# Autodesk Inventor assembly: robot base
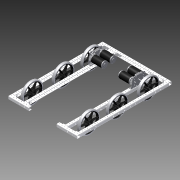
[picture p0: Inventor's stored thumbnail of the model, 180x180]
Saved by Autodesk Inventor 2011 SP1 (Build 150282100, 282)
## iProperties
Created: 2012-01-19
Part Number: robot base
Document SubType Name: Assembly
Designer: Christopher
Author: Christopher
## Documents named in this file (7)
- C:\Users\Christopher\Documents\Christopher\FIRST\Inventor files\2012\robot base.iam
- C:\Users\Christopher\Documents\Christopher\FIRST\Inventor files\2011\Kit of Parts\Chassis\Chassis_CornerConnect_AndyMark_am-0212.ipt
- C:\Users\Christopher\Documents\Christopher\FIRST\Inventor files\2011\Kit of Parts\Chassis\Chassis_CIMGearbox_AndyMark_am-0734.ipt
- C:\Users\Christopher\Documents\Christopher\FIRST\Inventor files\2011\Kit of Parts\Chassis\Chassis_Channel_AndyMark_am-0202.ipt
- C:\Users\Christopher\Documents\Christopher\FIRST\Inventor files\2011\Kit of Parts\Chassis\Chassis_Wheel_AndyMark_am-0420.iam
- C:\Users\Christopher\Documents\Christopher\FIRST\Inventor files\2011\Kit of Parts\Chassis\chassis 27 inch.ipt
- C:\Users\Christopher\Documents\Christopher\FIRST\Inventor files\2011\Kit of Parts\Chassis\chassis 9 inch.ipt
## Components (23 placed, 6 different names)
1. Chassis_CornerConnect_AndyMark_am-0212:1 — Insert:3, Insert:4, Insert:30
2. Chassis_CornerConnect_AndyMark_am-0212:4 — Insert:22, Insert:23, Insert:26, Insert:27
3. Chassis_CornerConnect_AndyMark_am-0212:5 — Insert:13, Insert:14, Insert:31
4. Chassis_CornerConnect_AndyMark_am-0212:6 — Insert:7, Insert:8
5. Chassis_CornerConnect_AndyMark_am-0212:7 — Insert:1, Insert:2, Insert:5, Insert:6
6. Chassis_CornerConnect_AndyMark_am-0212:8 — Insert:9, Insert:10, Insert:11, Insert:12
7. Chassis_CornerConnect_AndyMark_am-0212:9 — Insert:28, Insert:32
8. Chassis_CornerConnect_AndyMark_am-0212:10 — Insert:20, Insert:21, Insert:29
9. Chassis_CIMGearbox_AndyMark_am-0734:1 — Insert:35, Insert:36
10. Chassis_CIMGearbox_AndyMark_am-0734:2 — Insert:33, Insert:34
11. Chassis_Channel_AndyMark_am-0202:1 — Insert:11, Insert:12, Insert:13, Insert:14, Insert:37, Insert:38, Insert:39
12. Chassis_Channel_AndyMark_am-0202:3 — Insert:1, Insert:2, Insert:3, Insert:4, Insert:40, Insert:42, Insert:43
13. Chassis_Channel_AndyMark_am-0202:4 — Insert:26, Insert:27, Insert:28, Insert:33, Insert:34
14. Chassis_Channel_AndyMark_am-0202:5 — Insert:20, Insert:21, Insert:35, Insert:36
15. Chassis_Wheel_AndyMark_am-0420:1 [sub-assembly] — Insert:40
16. Chassis_Wheel_AndyMark_am-0420:2 [sub-assembly] — Insert:42
17. Chassis_Wheel_AndyMark_am-0420:3 [sub-assembly] — Insert:43
18. Chassis_Wheel_AndyMark_am-0420:4 [sub-assembly] — Insert:38
19. Chassis_Wheel_AndyMark_am-0420:5 [sub-assembly] — Insert:37
20. Chassis_Wheel_AndyMark_am-0420:6 [sub-assembly] — Insert:39
21. chassis 27 inch:1 — Insert:5, Insert:6, Insert:7, Insert:8, Insert:9, Insert:10, Insert:22, Insert:23
22. chassis 9 inch:1 — Insert:29, Insert:30
23. chassis 9 inch:2 — Insert:31, Insert:32
## Relationships (35: Insert 35)
- Insert:1: Chassis_CornerConnect_AndyMark_am-0212:7 ↔ Chassis_Channel_AndyMark_am-0202:3
- Insert:2: Chassis_CornerConnect_AndyMark_am-0212:7 ↔ Chassis_Channel_AndyMark_am-0202:3
- Insert:3: Chassis_CornerConnect_AndyMark_am-0212:1 ↔ Chassis_Channel_AndyMark_am-0202:3
- Insert:4: Chassis_CornerConnect_AndyMark_am-0212:1 ↔ Chassis_Channel_AndyMark_am-0202:3
- Insert:5: Chassis_CornerConnect_AndyMark_am-0212:7 ↔ chassis 27 inch:1
- Insert:6: Chassis_CornerConnect_AndyMark_am-0212:7 ↔ chassis 27 inch:1
- Insert:7: Chassis_CornerConnect_AndyMark_am-0212:6 ↔ chassis 27 inch:1
- Insert:8: Chassis_CornerConnect_AndyMark_am-0212:6 ↔ chassis 27 inch:1
- Insert:9: Chassis_CornerConnect_AndyMark_am-0212:8 ↔ chassis 27 inch:1
- Insert:10: Chassis_CornerConnect_AndyMark_am-0212:8 ↔ chassis 27 inch:1
- Insert:11: Chassis_CornerConnect_AndyMark_am-0212:8 ↔ Chassis_Channel_AndyMark_am-0202:1
- Insert:12: Chassis_CornerConnect_AndyMark_am-0212:8 ↔ Chassis_Channel_AndyMark_am-0202:1
- Insert:13: Chassis_CornerConnect_AndyMark_am-0212:5 ↔ Chassis_Channel_AndyMark_am-0202:1
- Insert:14: Chassis_CornerConnect_AndyMark_am-0212:5 ↔ Chassis_Channel_AndyMark_am-0202:1
- Insert:20: Chassis_CornerConnect_AndyMark_am-0212:10 ↔ Chassis_Channel_AndyMark_am-0202:5
- Insert:21: Chassis_CornerConnect_AndyMark_am-0212:10 ↔ Chassis_Channel_AndyMark_am-0202:5
- Insert:22: Chassis_CornerConnect_AndyMark_am-0212:4 ↔ chassis 27 inch:1
- Insert:23: Chassis_CornerConnect_AndyMark_am-0212:4 ↔ chassis 27 inch:1
- Insert:26: Chassis_CornerConnect_AndyMark_am-0212:4 ↔ Chassis_Channel_AndyMark_am-0202:4
- Insert:27: Chassis_CornerConnect_AndyMark_am-0212:4 ↔ Chassis_Channel_AndyMark_am-0202:4
- Insert:28: Chassis_CornerConnect_AndyMark_am-0212:9 ↔ Chassis_Channel_AndyMark_am-0202:4
- Insert:29: Chassis_CornerConnect_AndyMark_am-0212:10 ↔ chassis 9 inch:1
- Insert:30: Chassis_CornerConnect_AndyMark_am-0212:1 ↔ chassis 9 inch:1
- Insert:31: Chassis_CornerConnect_AndyMark_am-0212:5 ↔ chassis 9 inch:2
- Insert:32: Chassis_CornerConnect_AndyMark_am-0212:9 ↔ chassis 9 inch:2
- Insert:33: Chassis_CIMGearbox_AndyMark_am-0734:2 ↔ Chassis_Channel_AndyMark_am-0202:4
- Insert:34: Chassis_CIMGearbox_AndyMark_am-0734:2 ↔ Chassis_Channel_AndyMark_am-0202:4
- Insert:35: Chassis_CIMGearbox_AndyMark_am-0734:1 ↔ Chassis_Channel_AndyMark_am-0202:5
- Insert:36: Chassis_CIMGearbox_AndyMark_am-0734:1 ↔ Chassis_Channel_AndyMark_am-0202:5
- Insert:37 (57.15 mm): Chassis_Channel_AndyMark_am-0202:1 ↔ Chassis_Wheel_AndyMark_am-0420:5
- Insert:38 (57.15 mm): Chassis_Channel_AndyMark_am-0202:1 ↔ Chassis_Wheel_AndyMark_am-0420:4
- Insert:39 (57.15 mm): Chassis_Channel_AndyMark_am-0202:1 ↔ Chassis_Wheel_AndyMark_am-0420:6
- Insert:40 (57.15 mm): Chassis_Channel_AndyMark_am-0202:3 ↔ Chassis_Wheel_AndyMark_am-0420:1
- Insert:42 (57.15 mm): Chassis_Channel_AndyMark_am-0202:3 ↔ Chassis_Wheel_AndyMark_am-0420:2
- Insert:43 (57.15 mm): Chassis_Channel_AndyMark_am-0202:3 ↔ Chassis_Wheel_AndyMark_am-0420:3
